# Autodesk Inventor assembly: Base
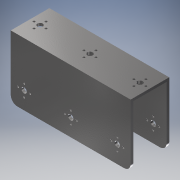
[picture p0: Inventor's stored thumbnail of the model, 180x180]
Saved by Autodesk Inventor 2018 (Build 220112000, 112)
## iProperties
Created: 2019-04-03
Part Number: Base
Material: Genérico
Document SubType Name: Assembly
Designer: Victor Hernandez
Author: Victor Hernandez
## Documents named in this file (3)
- C:\Users\Victor Hernandez\Desktop\Quinto Cuatrimestre\Garabito\robot\Base.iam
- C:\Users\Victor Hernandez\Desktop\Quinto Cuatrimestre\Garabito\robot\frontal2.ipt
- C:\Users\Victor Hernandez\Desktop\Quinto Cuatrimestre\Garabito\robot\laterales2.ipt
## Components (3 placed, 2 different names)
1. frontal2:1 — Coincidencia:1, Coincidencia:2, Coincidencia:3, Coincidencia:4
2. laterales2:1 — Coincidencia:1, Coincidencia:2
3. laterales2:2 — Coincidencia:3, Coincidencia:4
## Relationships (4: Mate 4)
- Coincidencia:1 [Mate]: frontal2:1 ↔ laterales2:1
- Coincidencia:2 [Mate]: frontal2:1 ↔ laterales2:1
- Coincidencia:3 [Mate]: frontal2:1 ↔ laterales2:2
- Coincidencia:4 [Mate]: frontal2:1 ↔ laterales2:2
